# Autodesk Inventor assembly: HACKberry_v1_for_print6
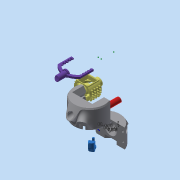
[picture p0: Inventor's stored thumbnail of the model, 180x180]
Saved by Autodesk Inventor 2016 (Build 200138000, 138)
## iProperties
Created: 2015-02-09
Part Number: HACKberry_v1_for_print6
Document SubType Name: Assembly
Designer: Yamaura
Author: Yamaura
## Documents named in this file (8)
- C:\Users\Hayato\Documents\exiii\hackberry\HACKberry-hardware\3D\Inventor\HACKberry_v1_for_print6.iam
- C:\Users\Hayato\Documents\exiii\hackberry\HACKberry-hardware\3D\Inventor\Parts\HBpronationLockPin02.ipt
- C:\Users\Hayato\Documents\exiii\hackberry\HACKberry-hardware\3D\Inventor\Parts\HBlockPlateHolder02.ipt
- C:\Users\Hayato\Documents\exiii\hackberry\HACKberry-hardware\3D\Inventor\Parts\HBabductionLever02.ipt
- C:\Users\Hayato\Documents\exiii\hackberry\HACKberry-hardware\3D\Inventor\Parts\HBejectorLever02.ipt
- C:\Users\Hayato\Documents\exiii\hackberry\HACKberry-hardware\3D\Inventor\Parts\HBarmMount02.ipt
- C:\Users\Hayato\Documents\exiii\hackberry\HACKberry-hardware\3D\Inventor\Parts\HBarmMountBaseCover03.ipt
- C:\Users\Hayato\Documents\exiii\hackberry\HACKberry-hardware\3D\Inventor\Parts\HBarmMountBase03.ipt
## Components (7 placed, 7 different names)
1. HBpronationLockPin02:1
2. HBlockPlateHolder02:1
3. HBarmMountBaseCover03:1
4. HBabductionLever02:1
5. HBejectorLever02:1
6. HBarmMount02:1
7. HBarmMountBase03:1 — メイト:76, フラッシュ:14
## Relationships (2: Mate 1, Flush 1)
- メイト:76 [Mate]: HBarmMountBase03:1
- フラッシュ:14 [Flush] (-9.2 mm): HBarmMountBase03:1
